# Autodesk Inventor assembly: motor
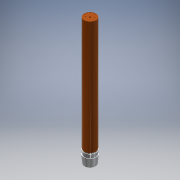
[picture p0: Inventor's stored thumbnail of the model, 180x180]
Saved by Autodesk Inventor 2017 SP1 (Build 210196100, 196)
## iProperties
Created: 2016-10-21
Part Number: motor
Document SubType Name: Assembly
Designer: cflannery
Author: cflannery
## Documents named in this file (4)
- D:\Triton_Rocket_Club\NONGIT\Vehicles\Intrepid\Structures\motor.iam
- D:\Triton_Rocket_Club\NONGIT\Vehicles\Intrepid\Nozzle\nozzle.iam
- D:\Triton_Rocket_Club\NONGIT\Vehicles\Intrepid\Structures\phenolic_liner.ipt
- D:\Triton_Rocket_Club\NONGIT\Vehicles\Intrepid\Structures\upper_thermal_barrier.ipt
## Components (3 placed, 3 different names)
1. phenolic_liner:1 — Mate:3, Mate:4, Mate:5, Mate:6
2. upper_thermal_barrier:1 — Mate:3, Mate:6
3. nozzle:1 [sub-assembly] — Mate:4, Mate:5
## Relationships (4: Mate 4)
- Mate:3: phenolic_liner:1 ↔ upper_thermal_barrier:1
- Mate:4: phenolic_liner:1 ↔ nozzle:1
- Mate:5: phenolic_liner:1 ↔ nozzle:1
- Mate:6: phenolic_liner:1 ↔ upper_thermal_barrier:1
